# Autodesk Inventor assembly: 2050
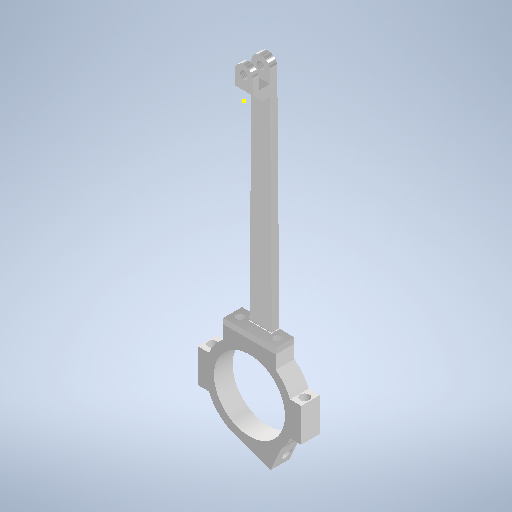
[picture p0: Inventor's stored thumbnail of the model, 512x512]
Saved by Autodesk Inventor 2025.1 (Build 291241000, 241)
## iProperties
Created: 2024-06-01
Part Number: 2050
Document SubType Name: Assembly
Designer: Fabri
Author: Fabri
## Documents named in this file (3)
- C:\Users\ffogue\Downloads\Meine Projket\Paddle\2050.iam
- C:\Users\ffogue\Downloads\Meine Projket\Paddle\2051.ipt
- C:\Users\ffogue\Downloads\Meine Projket\Paddle\205.ipt
## Components (2 placed, 2 different names)
1. 2051:1 — Mate:1, Mate:2, Insert:1
2. 205:1 — Mate:1, Mate:2, Insert:1, Angle:1
## Relationships (4: Mate 2, Insert 1, Angle 1)
- Mate:1: 2051:1 ↔ 205:1
- Mate:2: 2051:1 ↔ 205:1
- Insert:1: 2051:1 ↔ 205:1
- Angle:1 (0 deg): 205:1
